# Autodesk Inventor assembly: Standard (DIN)
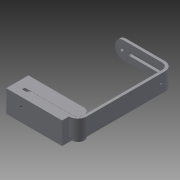
[picture p0: Inventor's stored thumbnail of the model, 180x180]
Saved by Autodesk Inventor 2014 (Build 180170000, 170)
## iProperties
Shininess: 64.0
Length Units: 11269
Angle Units: 11279
Time Units: 11290
Mass Units: 11283
Length Display Precision: 3
Angle Display Precision: 2
Compacted: True
Part Number: Standard (DIN)
Document SubType Name: Assembly
Density: 0.0
Volumn: 0.0
Area: 0.0
PropertySet Name: Model Information
Control State: 0
Master: False
Checked Out: False
## Documents named in this file (3)
- F:\projekte\Inventor\Projekte\Lampenkopf_v4\Biegetest.iam
- F:\projekte\Inventor\Projekte\Lampenkopf_v4\Biegehilfe.ipt
- F:\PROJEKTE\INVENTOR\PROJEKTE\LAMPENKOPF_V4\Haltegriff.ipt
## Components (2 placed, 2 different names)
1. Biegehilfe:1 — Starr:1
2. Haltegriff:1 — Starr:1
## Relationships (1: WeldJoint 1)
- Starr:1 [WeldJoint]: Biegehilfe:1 ↔ Haltegriff:1
